# Autodesk Inventor assembly: Linear Gripper
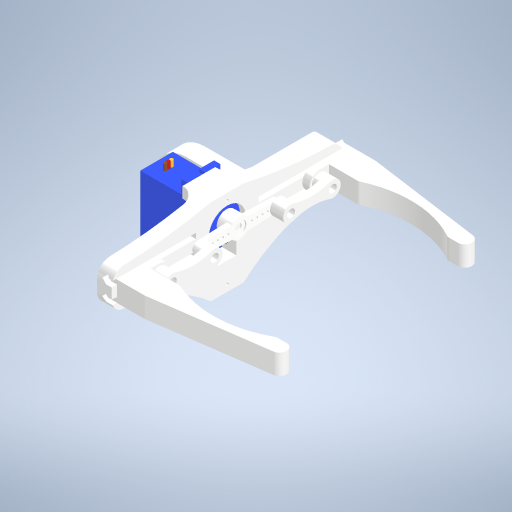
[picture p0: Inventor's stored thumbnail of the model, 512x512]
Saved by Autodesk Inventor 2024 (Build 280153000, 153)
## iProperties
Created: 2020-06-18
Part Number: Linear Gripper
Document SubType Name: Assembly
Designer: jebes windows
Sending System: SolidWorks 2019
Last Author: jason
Last Saved: 2020-08-17
Author: jebes windows
## Documents named in this file (7)
- C:\Users\jebes windows\Documents\Inventor\Robotska_roka\linear-gripper-1.snapshot.4\Linear Gripper\Linear Gripper.iam
- C:\Users\jebes windows\Documents\Inventor\Robotska_roka\linear-gripper-1.snapshot.4\Linear Gripper\Linear Base.ipt
- C:\Users\jebes windows\Documents\Inventor\Robotska_roka\linear-gripper-1.snapshot.4\Linear Gripper\Servo Micro.ipt
- C:\Users\jebes windows\Documents\Inventor\Robotska_roka\linear-gripper-1.snapshot.4\Linear Gripper\Horn.ipt
- C:\Users\jebes windows\Documents\Inventor\Robotska_roka\linear-gripper-1.snapshot.4\Linear Gripper\LGrip.ipt
- C:\Users\jebes windows\Documents\Inventor\Robotska_roka\linear-gripper-1.snapshot.4\Linear Gripper\Linear Link.ipt
- C:\Users\jebes windows\Documents\Inventor\Robotska_roka\linear-gripper-1.snapshot.4\Linear Gripper\LGrip Mirror.ipt
## Components (7 placed, 6 different names)
1. Linear Base:1 — Mate:1, Mate:2, Flush:1, Mate:10, Mate:13
2. Servo Micro:2 — Insert:1, Mate:1, Mate:2, Flush:1
3. Horn:1 — Insert:1, Mate:4, Mate:6, Mate:7, Mate:9, Tangent:1
4. LGrip:1 — Mate:8, Mate:12, Mate:13
5. Linear Link:1 — Mate:6, Mate:7, Mate:8, Mate:12
6. Linear Link:2 — Mate:4, Mate:5, Mate:9, Mate:11
7. LGrip Mirror:1 — Mate:5, Mate:10, Mate:11, Tangent:1
## Relationships (15: Mate 12, Insert 1, Flush 1, Tangent 1)
- Insert:1: Servo Micro:2 ↔ Horn:1
- Mate:1: Linear Base:1 ↔ Servo Micro:2
- Mate:2: Linear Base:1 ↔ Servo Micro:2
- Flush:1: Linear Base:1 ↔ Servo Micro:2
- Mate:4: Horn:1 ↔ Linear Link:2
- Mate:5: Linear Link:2 ↔ LGrip Mirror:1
- Mate:6: Horn:1 ↔ Linear Link:1
- Mate:7: Horn:1 ↔ Linear Link:1
- Mate:8: LGrip:1 ↔ Linear Link:1
- Mate:9: Horn:1 ↔ Linear Link:2
- Mate:10: Linear Base:1 ↔ LGrip Mirror:1
- Mate:11: Linear Link:2 ↔ LGrip Mirror:1
- Mate:12: LGrip:1 ↔ Linear Link:1
- Mate:13: Linear Base:1 ↔ LGrip:1
- Tangent:1: Horn:1 ↔ LGrip Mirror:1
